# Autodesk Inventor assembly: X_Carriage_V2_0
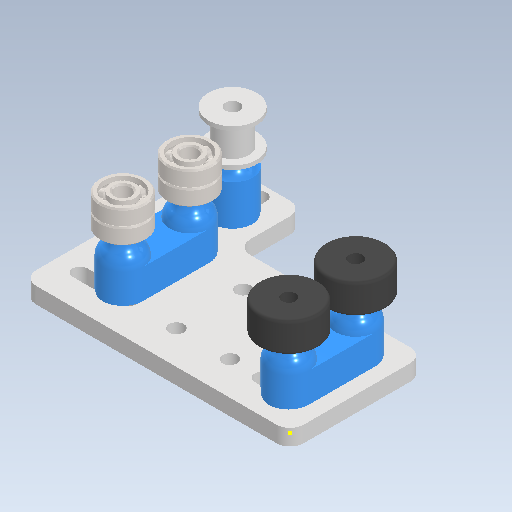
[picture p0: Inventor's stored thumbnail of the model, 512x512]
Saved by Autodesk Inventor 2021 (Build 250183000, 183)
## iProperties
Created: 2021-06-13
Part Number: X_Carriage_V2_0
Document SubType Name: Assembly
Designer: Jorian Brusind
Author: Jorian Brusind
## Documents named in this file (7)
- C:\Users\Jorian Bruslind\Documents\GitHub\PersonalProjects\HyperRail\Inventor Files\X_Carriage_V2_0.iam
- C:\Users\Jorian Bruslind\Documents\GitHub\PersonalProjects\HyperRail\Inventor Files\X_Carriage_Plate.ipt
- C:\Users\Jorian Bruslind\Documents\GitHub\PersonalProjects\HyperRail\Inventor Files\11mm_BearingWheel.ipt
- C:\Users\Jorian Bruslind\Documents\GitHub\PersonalProjects\HyperRail\Inventor Files\4mm_Roller_Spacer_simple.ipt
- C:\Users\Jorian Bruslind\Documents\GitHub\PersonalProjects\HyperRail\Inventor Files\Rollder_Spacer_Single.ipt
- C:\Users\Jorian Bruslind\Documents\GitHub\PersonalProjects\HyperRail\Inventor Files\10mm_Idle_Pulley.ipt
- C:\Users\Jorian Bruslind\Documents\GitHub\PersonalProjects\HyperRail\Inventor Files\606zz_bearing.ipt
## Components (11 placed, 6 different names)
1. X_Carriage_Plate:1 — Mate:1, Mate:2, Mate:7, Mate:14, Mate:27, Mate:29, Mate:31, Mate:32, Mate:33, Mate:42, Angle:1
2. 11mm_BearingWheel:1 — Mate:1, Flush:2
3. 11mm_BearingWheel:4 — Mate:2, Flush:2, Mate:7
4. 4mm_Roller_Spacer_simple:2 — Mate:14, Mate:39, Mate:40, Mate:41, Mate:42, Angle:1
5. Rollder_Spacer_Single:1 — Mate:27, Mate:28, Mate:29, Mate:30
6. 10mm_Idle_Pulley:1 — Mate:28, Mate:30
7. 4mm_Roller_Spacer_simple:3 — Mate:31, Mate:32, Mate:33
8. 606zz_bearing:1 — Mate:35, Mate:37, Flush:3, Mate:40
9. 606zz_bearing:2 — Mate:35, Mate:37, Mate:41
10. 606zz_bearing:3 — Mate:34, Mate:36, Flush:3
11. 606zz_bearing:4 — Mate:34, Mate:36, Mate:39
## Relationships (22: Mate 19, Flush 2, Angle 1)
- Mate:1: X_Carriage_Plate:1 ↔ 11mm_BearingWheel:1
- Mate:2: X_Carriage_Plate:1 ↔ 11mm_BearingWheel:4
- Flush:2: 11mm_BearingWheel:1 ↔ 11mm_BearingWheel:4
- Mate:7 (20 mm): X_Carriage_Plate:1 ↔ 11mm_BearingWheel:4
- Mate:14: X_Carriage_Plate:1 ↔ 4mm_Roller_Spacer_simple:2
- Mate:27: X_Carriage_Plate:1 ↔ Rollder_Spacer_Single:1
- Mate:28: Rollder_Spacer_Single:1 ↔ 10mm_Idle_Pulley:1
- Mate:29: X_Carriage_Plate:1 ↔ Rollder_Spacer_Single:1
- Mate:30: Rollder_Spacer_Single:1 ↔ 10mm_Idle_Pulley:1
- Mate:31: X_Carriage_Plate:1 ↔ 4mm_Roller_Spacer_simple:3
- Mate:32: X_Carriage_Plate:1 ↔ 4mm_Roller_Spacer_simple:3
- Mate:33: X_Carriage_Plate:1 ↔ 4mm_Roller_Spacer_simple:3
- Mate:34: 606zz_bearing:3 ↔ 606zz_bearing:4
- Mate:35: 606zz_bearing:1 ↔ 606zz_bearing:2
- Mate:36: 606zz_bearing:3 ↔ 606zz_bearing:4
- Mate:37: 606zz_bearing:1 ↔ 606zz_bearing:2
- Mate:39: 4mm_Roller_Spacer_simple:2 ↔ 606zz_bearing:4
- Flush:3: 606zz_bearing:1 ↔ 606zz_bearing:3
- Mate:40: 4mm_Roller_Spacer_simple:2 ↔ 606zz_bearing:1
- Mate:41: 4mm_Roller_Spacer_simple:2 ↔ 606zz_bearing:2
- Mate:42 (-15 mm): X_Carriage_Plate:1 ↔ 4mm_Roller_Spacer_simple:2
- Angle:1 (0 deg): X_Carriage_Plate:1 ↔ 4mm_Roller_Spacer_simple:2
